# Autodesk Inventor assembly: horizontal_stabilizer
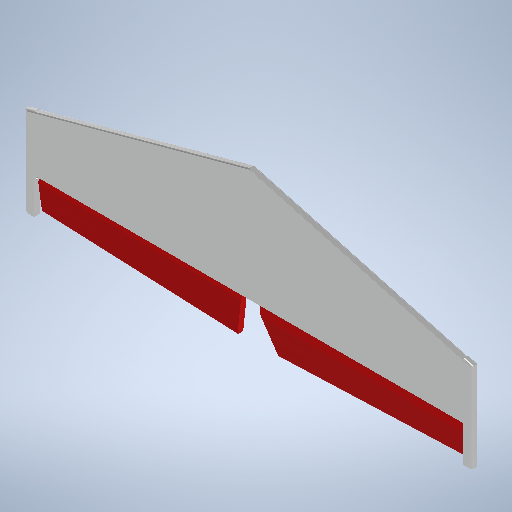
[picture p0: Inventor's stored thumbnail of the model, 512x512]
Saved by Autodesk Inventor 2025.3 (Build 293356000, 356)
## iProperties
Created: 2025-07-09
Part Number: horizontal_stabilizer
Document SubType Name: Assembly
Designer: steve
Author: steve
## Documents named in this file (4)
- C:\Users\steve\OneDrive\Documentos\Avion\MODELOS NUEVOS\HORIZONTAL STABILIZER\horizontal_stabilizer.iam
- C:\Users\steve\OneDrive\Documentos\Avion\MODELOS NUEVOS\HORIZONTAL STABILIZER\Part1.ipt
- C:\Users\steve\OneDrive\Documentos\Avion\MODELOS NUEVOS\HORIZONTAL STABILIZER\Part11.ipt
- C:\Users\steve\OneDrive\Documentos\Avion\MODELOS NUEVOS\HORIZONTAL STABILIZER\Part12.ipt
## Components (3 placed, 3 different names)
1. Part1:1 — Rotational:1, Rotational:2
2. Part11:1 — Rotational:2
3. Part12:1 — Rotational:1
## Relationships (2: RevoluteJoint 2)
- Rotational:1 [RevoluteJoint] (-99 mm): Part1:1 ↔ Part12:1
- Rotational:2 [RevoluteJoint] (10 mm): Part1:1 ↔ Part11:1
## Named parameters: Finish1_Area = 1093.06, Finish1_Thickness = 0.008 mm, Finish2_Area = 302.075, Finish3_Area = 12.9954
note: some values were not read from the file. Shown as the stored number, unit unknown: "Finish1_Area", "Finish2_Area", "Finish3_Area".
